# Autodesk Inventor assembly: MainAssembly
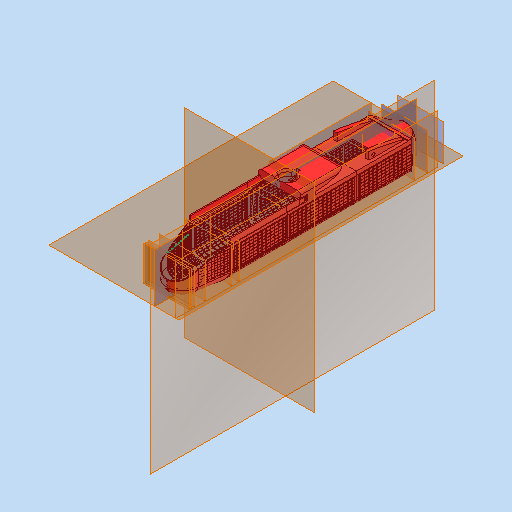
[picture p0: Inventor's stored thumbnail of the model, 512x512]
Saved by Autodesk Inventor 2027 (Build 310192060, 192F)
## iProperties
Created: 2026-09-14
Part Number: MainAssembly
Document SubType Name: Assembly
Designer: mateo
Author: mateo
## Documents named in this file (2)
- C:\GitHub\SWIFT-UAV\System_development\Pelican\structural_model\v0.3.1\MainAssembly\MainAssembly.iam
- C:\GitHub\SWIFT-UAV\System_development\Pelican\structural_model\v0.3.1\Parts\Fuselage\FuselageV2.ipt
## Components (1 placed, 1 different names)
1. FuselageV2:1 — Mate:1, Mate:2, Mate:3
## Relationships (3: Mate 3)
- Mate:1: FuselageV2:1
- Mate:2 (-428.1297 mm): FuselageV2:1
- Mate:3: FuselageV2:1
